# Autodesk Inventor assembly: UpperArm
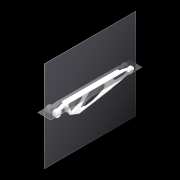
[picture p0: Inventor's stored thumbnail of the model, 180x180]
Saved by Autodesk Inventor 2020.5 (Build 245400000, 400)
## iProperties
Created: 2023-03-17
Part Number: UpperArm
Document SubType Name: Assembly
Designer: valer
Author: valer
## Documents named in this file (2)
- C:\Users\valer\Desktop\urdf-export\UpperArm.iam
- C:\Users\valer\Desktop\drummingrobot\src\parts\UpperArm.ipt
## Components (1 placed, 1 different names)
1. UpperArm:1 — Mate:1, Angle:1, Mate:2
## Relationships (3: Mate 2, Angle 1)
- Mate:1: UpperArm:1
- Angle:1 (0 deg): UpperArm:1
- Mate:2: UpperArm:1
